# Autodesk Inventor assembly: HeadUnit
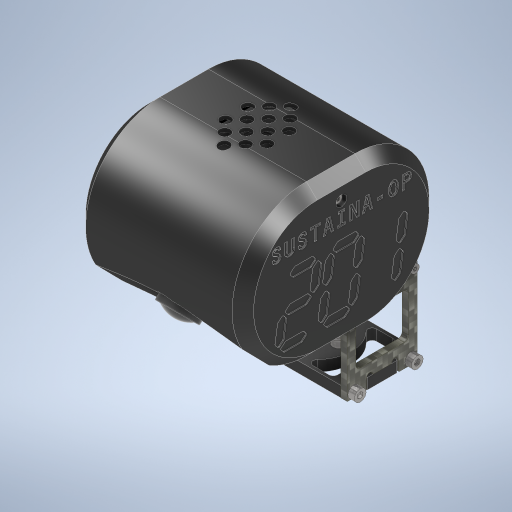
[picture p0: Inventor's stored thumbnail of the model, 512x512]
Saved by Autodesk Inventor 2024.2 (Build 282272000, 272)
## iProperties
Created: 2024-01-19
Part Number: HeadUnit
Document SubType Name: Assembly
Designer: Masato Kubotera
Mass: 257.797 g
Surface Area: 969.022 cm^2
Volume: 207.363 cm^3
Density: 1.24322 g/cm^3
Author: Masato Kubotera
## Documents named in this file (22)
- C:\Users\masato\OneDrive - Chiba Institute of Technology\CIT Brains\RoboCup2024\SUSTAINA-OP2-DEV\NativeFiles\Boby\Head\HeadUnit.iam
- C:\Users\masato\OneDrive - Chiba Institute of Technology\CIT Brains\RoboCup2024\SUSTAINA-OP2-DEV\NativeFiles\Boby\COTS\Screws\CapScrew\UC-0308.ipt
- C:\Users\masato\OneDrive - Chiba Institute of Technology\CIT Brains\RoboCup2024\SUSTAINA-OP2-DEV\NativeFiles\Boby\Head\HeadCameraMountFrame.ipt
- C:\Users\masato\OneDrive - Chiba Institute of Technology\CIT Brains\RoboCup2024\SUSTAINA-OP2-DEV\NativeFiles\Boby\Head\HeadHornFrame.ipt
- C:\Users\masato\OneDrive - Chiba Institute of Technology\CIT Brains\RoboCup2024\SUSTAINA-OP2-DEV\NativeFiles\Boby\COTS\Spacers\C-2006-4.ipt
- C:\Users\masato\OneDrive - Chiba Institute of Technology\CIT Brains\RoboCup2024\SUSTAINA-OP2-DEV\NativeFiles\Boby\COTS\ElectronicComponents\CMS-402811-28SP.ipt
- C:\Users\masato\OneDrive - Chiba Institute of Technology\CIT Brains\RoboCup2024\SUSTAINA-OP2-DEV\NativeFiles\Boby\COTS\Screws\CapScrew\UC-0206.ipt
- C:\Users\masato\OneDrive - Chiba Institute of Technology\CIT Brains\RoboCup2024\SUSTAINA-OP2-DEV\NativeFiles\Boby\COTS\ElectronicComponents\Cameras\e-CAM50_CUONX.ipt
- C:\Users\masato\OneDrive - Chiba Institute of Technology\CIT Brains\RoboCup2024\SUSTAINA-OP2-DEV\NativeFiles\Boby\COTS\Spacers\C-2002.5-4.ipt
- C:\Users\masato\OneDrive - Chiba Institute of Technology\CIT Brains\RoboCup2024\SUSTAINA-OP2-DEV\NativeFiles\Boby\COTS\Screws\CapScrew\FC-0215EB.ipt
- C:\Users\masato\OneDrive - Chiba Institute of Technology\CIT Brains\RoboCup2024\SUSTAINA-OP2-DEV\NativeFiles\Boby\COTS\CIL926-F2.4-M12A650.ipt
- C:\Users\masato\OneDrive - Chiba Institute of Technology\CIT Brains\RoboCup2024\SUSTAINA-OP2-DEV\NativeFiles\Boby\COTS\ElectronicComponents\SEN0539-EN.ipt
- C:\Users\masato\OneDrive - Chiba Institute of Technology\CIT Brains\RoboCup2024\SUSTAINA-OP2-DEV\NativeFiles\Boby\CustomPCBs\SUSTAINA-SCI-EXTENSION-BORAD.ipt
- C:\Users\masato\OneDrive - Chiba Institute of Technology\CIT Brains\RoboCup2024\SUSTAINA-OP2-DEV\NativeFiles\Boby\CustomPCBs\SUSTAINA-AUDIO-BOARD.ipt
- C:\Users\masato\OneDrive - Chiba Institute of Technology\CIT Brains\RoboCup2024\SUSTAINA-OP2-DEV\NativeFiles\Boby\Head\HeadUpperFrame.ipt
- C:\Users\masato\OneDrive - Chiba Institute of Technology\CIT Brains\RoboCup2024\SUSTAINA-OP2-DEV\NativeFiles\Boby\COTS\Screws\LowHeadCapScrew\ULC-0308.ipt
- C:\Users\masato\OneDrive - Chiba Institute of Technology\CIT Brains\RoboCup2024\SUSTAINA-OP2-DEV\NativeFiles\Boby\COTS\Spacers\WBN-305.ipt
- C:\Users\masato\OneDrive - Chiba Institute of Technology\CIT Brains\RoboCup2024\SUSTAINA-OP2-DEV\NativeFiles\Boby\Head\HeadLowerFrame.ipt
- C:\Users\masato\OneDrive - Chiba Institute of Technology\CIT Brains\RoboCup2024\SUSTAINA-OP2-DEV\NativeFiles\Boby\COTS\Screws\CapScrew\UC-0306.ipt
- C:\Users\masato\OneDrive - Chiba Institute of Technology\CIT Brains\RoboCup2024\SUSTAINA-OP2-DEV\NativeFiles\Boby\Head\HeadSideFrame.ipt
- C:\Users\masato\OneDrive - Chiba Institute of Technology\CIT Brains\RoboCup2024\SUSTAINA-OP2-DEV\NativeFiles\Boby\Head\HeadCover.ipt
- C:\Users\masato\OneDrive - Chiba Institute of Technology\CIT Brains\RoboCup2024\SUSTAINA-OP2-DEV\NativeFiles\Boby\COTS\Screws\CapScrew\UC-0210.ipt
## Components (56 placed, 21 different names)
1. HeadUpperFrame:1 — Insert:127, Insert:128, Insert:133, Insert:134, Insert:135, Insert:136, Insert:173, Insert:174
2. HeadLowerFrame:1 — Insert:94, Insert:95, Insert:141, Insert:142, Insert:169, Insert:170, Insert:171, Insert:172
3. HeadCameraMountFrame:1 — Insert:92, Insert:93, Insert:157, Insert:158, Insert:159, Insert:160
4. HeadHornFrame:1 — Mate:1, Angle:1, Mate:2, Insert:24, Insert:25, Insert:26, Insert:145, Insert:146, Insert:149, Insert:150
5. HeadSideFrame:1 — Insert:145, Insert:146, Insert:147, Insert:148, Insert:153, Insert:154, Insert:157, Insert:158, Insert:163, Insert:164, Insert:165, Insert:166, Insert:169, Insert:170, Insert:173, Insert:174
6. HeadSideFrame:2 — Insert:149, Insert:150, Insert:151, Insert:152, Insert:155, Insert:156, Insert:159, Insert:160, Insert:161, Insert:162, Insert:167, Insert:168, Insert:171, Insert:172
7. SUSTAINA-AUDIO-BOARD:1 — Insert:137, Insert:138, Insert:139, Insert:140
8. SUSTAINA-SCI-EXTENSION-BORAD:1 — Insert:94, Insert:95, Insert:96, Insert:97
9. HeadCover:1 — Flush:5, Flush:6, Flush:7, Insert:175, Insert:176
10. CIL926-F2.4-M12A650:1 — Mate:119, Flush:4
11. SEN0539-EN:1 — Insert:141, Insert:142, Insert:143, Insert:144
12. CMS-402811-28SP:1 — Insert:127, Insert:128, Insert:129, Insert:130
13. e-CAM50_CUONX:1 — Insert:108, Insert:109, Insert:110, Insert:111, Insert:112, Insert:113, Insert:114, Insert:115, Insert:116, Insert:117, Mate:119, Insert:119, Insert:120, Flush:4
14. UC-0306:1 — Insert:143
15. UC-0306:2 — Insert:144
16. FC-0215EB:1 — Insert:108
17. FC-0215EB:2 — Insert:110
18. FC-0215EB:3 — Insert:112
19. FC-0215EB:4 — Insert:114
20. UC-0308:1 — Insert:147
21. UC-0308:2 — Insert:148
22. UC-0308:3 — Insert:152
23. UC-0308:4 — Insert:151
24. UC-0308:6 — Insert:24
25. UC-0308:7 — Insert:25
26. UC-0308:8 — Insert:26
27. ULC-0308:1 — Insert:130
28. ULC-0308:2 — Insert:129
29. UC-0206:3 — Insert:163
30. UC-0206:4 — Insert:164
31. UC-0206:5 — Insert:166
32. UC-0206:6 — Insert:165
33. UC-0206:7 — Insert:161
34. UC-0206:8 — Insert:162
35. UC-0206:9 — Insert:168
36. UC-0206:10 — Insert:167
37. UC-0206:11 — Insert:153
38. UC-0206:12 — Insert:154
39. UC-0206:13 — Insert:155
40. UC-0206:14 — Insert:156
41. UC-0206:15 — Insert:96
42. UC-0206:16 — Insert:97
43. UC-0210:1 — Insert:175
44. UC-0210:2 — Insert:176
45. WBN-305:1 — Insert:133, Insert:137
46. WBN-305:2 — Insert:134, Insert:139
47. WBN-305:3 — Insert:135, Insert:138
48. WBN-305:4 — Insert:136, Insert:140
49. C-2006-4:1 — Insert:109
50. C-2006-4:2 — Insert:113
51. C-2006-4:3 — Insert:111
52. C-2006-4:4 — Insert:115
53. C-2002.5-4:1 — Insert:93, Insert:116
54. C-2002.5-4:2 — Insert:92, Insert:117
55. C-2002.5-4:3 — Insert:119
56. C-2002.5-4:4 — Insert:120
## Relationships (77: Insert 69, Flush 4, Mate 3, Angle 1)
- Mate:1: HeadHornFrame:1
- Angle:1 (0 deg): HeadHornFrame:1
- Mate:2: HeadHornFrame:1
- Insert:24: HeadHornFrame:1 ↔ UC-0308:6
- Insert:25: HeadHornFrame:1 ↔ UC-0308:7
- Insert:26: HeadHornFrame:1 ↔ UC-0308:8
- Insert:92: HeadCameraMountFrame:1 ↔ C-2002.5-4:2
- Insert:93: HeadCameraMountFrame:1 ↔ C-2002.5-4:1
- Insert:94: HeadLowerFrame:1 ↔ SUSTAINA-SCI-EXTENSION-BORAD:1
- Insert:95: HeadLowerFrame:1 ↔ SUSTAINA-SCI-EXTENSION-BORAD:1
- Insert:96: SUSTAINA-SCI-EXTENSION-BORAD:1 ↔ UC-0206:15
- Insert:97: SUSTAINA-SCI-EXTENSION-BORAD:1 ↔ UC-0206:16
- Insert:108: e-CAM50_CUONX:1 ↔ FC-0215EB:1
- Insert:109: e-CAM50_CUONX:1 ↔ C-2006-4:1
- Insert:110: e-CAM50_CUONX:1 ↔ FC-0215EB:2
- Insert:111: e-CAM50_CUONX:1 ↔ C-2006-4:3
- Insert:112: e-CAM50_CUONX:1 ↔ FC-0215EB:3
- Insert:113: e-CAM50_CUONX:1 ↔ C-2006-4:2
- Insert:114: e-CAM50_CUONX:1 ↔ FC-0215EB:4
- Insert:115: e-CAM50_CUONX:1 ↔ C-2006-4:4
- Insert:116: e-CAM50_CUONX:1 ↔ C-2002.5-4:1
- Insert:117: e-CAM50_CUONX:1 ↔ C-2002.5-4:2
- Mate:119: CIL926-F2.4-M12A650:1 ↔ e-CAM50_CUONX:1
- Insert:119: e-CAM50_CUONX:1 ↔ C-2002.5-4:3
- Insert:120: e-CAM50_CUONX:1 ↔ C-2002.5-4:4
- Flush:4 (-23 mm): CIL926-F2.4-M12A650:1 ↔ e-CAM50_CUONX:1
- Insert:127: HeadUpperFrame:1 ↔ CMS-402811-28SP:1
- Insert:128: HeadUpperFrame:1 ↔ CMS-402811-28SP:1
- Insert:129: CMS-402811-28SP:1 ↔ ULC-0308:2
- Insert:130: CMS-402811-28SP:1 ↔ ULC-0308:1
- Insert:133: HeadUpperFrame:1 ↔ WBN-305:1
- Insert:134: HeadUpperFrame:1 ↔ WBN-305:2
- Insert:135: HeadUpperFrame:1 ↔ WBN-305:3
- Insert:136: HeadUpperFrame:1 ↔ WBN-305:4
- Insert:137: SUSTAINA-AUDIO-BOARD:1 ↔ WBN-305:1
- Insert:138: SUSTAINA-AUDIO-BOARD:1 ↔ WBN-305:3
- Insert:139: SUSTAINA-AUDIO-BOARD:1 ↔ WBN-305:2
- Insert:140: SUSTAINA-AUDIO-BOARD:1 ↔ WBN-305:4
- Insert:141: HeadLowerFrame:1 ↔ SEN0539-EN:1
- Insert:142: HeadLowerFrame:1 ↔ SEN0539-EN:1
- Insert:143: SEN0539-EN:1 ↔ UC-0306:1
- Insert:144: SEN0539-EN:1 ↔ UC-0306:2
- Insert:145: HeadHornFrame:1 ↔ HeadSideFrame:1
- Insert:146: HeadHornFrame:1 ↔ HeadSideFrame:1
- Insert:147: HeadSideFrame:1 ↔ UC-0308:1
- Insert:148: HeadSideFrame:1 ↔ UC-0308:2
- Insert:149: HeadHornFrame:1 ↔ HeadSideFrame:2
- Insert:150: HeadHornFrame:1 ↔ HeadSideFrame:2
- Insert:151: HeadSideFrame:2 ↔ UC-0308:4
- Insert:152: HeadSideFrame:2 ↔ UC-0308:3
- Insert:153: HeadSideFrame:1 ↔ UC-0206:11
- Insert:154: HeadSideFrame:1 ↔ UC-0206:12
- Insert:155: HeadSideFrame:2 ↔ UC-0206:13
- Insert:156: HeadSideFrame:2 ↔ UC-0206:14
- Insert:157: HeadCameraMountFrame:1 ↔ HeadSideFrame:1
- Insert:158: HeadCameraMountFrame:1 ↔ HeadSideFrame:1
- Insert:159: HeadCameraMountFrame:1 ↔ HeadSideFrame:2
- Insert:160: HeadCameraMountFrame:1 ↔ HeadSideFrame:2
- Insert:161: HeadSideFrame:2 ↔ UC-0206:7
- Insert:162: HeadSideFrame:2 ↔ UC-0206:8
- Insert:163: HeadSideFrame:1 ↔ UC-0206:3
- Insert:164: HeadSideFrame:1 ↔ UC-0206:4
- Insert:165: HeadSideFrame:1 ↔ UC-0206:6
- Insert:166: HeadSideFrame:1 ↔ UC-0206:5
- Insert:167: HeadSideFrame:2 ↔ UC-0206:10
- Insert:168: HeadSideFrame:2 ↔ UC-0206:9
- Insert:169: HeadLowerFrame:1 ↔ HeadSideFrame:1
- Insert:170: HeadLowerFrame:1 ↔ HeadSideFrame:1
- Insert:171: HeadLowerFrame:1 ↔ HeadSideFrame:2
- Insert:172: HeadLowerFrame:1 ↔ HeadSideFrame:2
- Flush:5: HeadCover:1
- Flush:6: HeadCover:1
- Flush:7: HeadCover:1
- Insert:173: HeadUpperFrame:1 ↔ HeadSideFrame:1
- Insert:174: HeadUpperFrame:1 ↔ HeadSideFrame:1
- Insert:175: HeadCover:1 ↔ UC-0210:1
- Insert:176: HeadCover:1 ↔ UC-0210:2
